# Autodesk Inventor assembly: Gantry
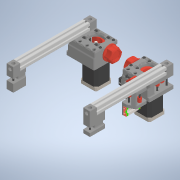
[picture p0: Inventor's stored thumbnail of the model, 180x180]
Saved by Autodesk Inventor 2022 (Build 260153000, 153)
## iProperties
Created: 2021-11-24
Part Number: Gantry
Document SubType Name: Assembly
Designer: yuto6
Author: yuto6
## Documents named in this file (7)
- C:\Users\yuto6\Documents\My3DPrinter\CAD\Asm\Gantry.iam
- C:\Users\yuto6\Documents\My3DPrinter\CAD\Parts\A_Idler (1).step.iam
- C:\Users\yuto6\Documents\My3DPrinter\CAD\Parts\B_Idler (1).step.iam
- C:\Users\yuto6\Documents\My3DPrinter\CAD\Parts\HFS3-1515-150.ipt
- C:\Users\yuto6\Documents\My3DPrinter\CAD\Parts\A_Drive.iam
- C:\Users\yuto6\Documents\My3DPrinter\CAD\Parts\B_Drive.iam
- C:\Users\yuto6\Documents\My3DPrinter\CAD\Parts\XY_Joint_Right.step.iam
## Components (7 placed, 6 different names)
1. B_Idler (1).step:1 [sub-assembly] — フラッシュ:1, フラッシュ:2, フラッシュ:3, メイト:1, メイト:2, メイト:5
2. A_Idler (1).step:1 [sub-assembly] — フラッシュ:1, フラッシュ:2, フラッシュ:4, メイト:3, メイト:4, メイト:5
3. HFS3-1515-150:1 — フラッシュ:3, メイト:1, メイト:2, メイト:8, メイト:9, フラッシュ:6
4. HFS3-1515-150:2 — フラッシュ:4, メイト:3, メイト:4, メイト:6, フラッシュ:5, メイト:7
5. A_Drive:1 [sub-assembly] — メイト:6, フラッシュ:5, メイト:7, フラッシュ:7, フラッシュ:8
6. B_Drive:1 [sub-assembly] — メイト:8, メイト:9, フラッシュ:6
7. XY_Joint_Right.step:1 [sub-assembly] — フラッシュ:7, フラッシュ:8
## Relationships (17: Mate 9, Flush 8)
- フラッシュ:1 [Flush]: B_Idler (1).step:1 ↔ A_Idler (1).step:1
- フラッシュ:2 [Flush]: B_Idler (1).step:1 ↔ A_Idler (1).step:1
- フラッシュ:3 [Flush]: B_Idler (1).step:1 ↔ HFS3-1515-150:1
- メイト:1 [Mate]: B_Idler (1).step:1 ↔ HFS3-1515-150:1
- メイト:2 [Mate]: B_Idler (1).step:1 ↔ HFS3-1515-150:1
- フラッシュ:4 [Flush]: A_Idler (1).step:1 ↔ HFS3-1515-150:2
- メイト:3 [Mate]: A_Idler (1).step:1 ↔ HFS3-1515-150:2
- メイト:4 [Mate]: A_Idler (1).step:1 ↔ HFS3-1515-150:2
- メイト:5 [Mate] (150 mm): B_Idler (1).step:1 ↔ A_Idler (1).step:1
- メイト:6 [Mate]: HFS3-1515-150:2 ↔ A_Drive:1
- フラッシュ:5 [Flush]: HFS3-1515-150:2 ↔ A_Drive:1
- メイト:7 [Mate]: HFS3-1515-150:2 ↔ A_Drive:1
- メイト:8 [Mate]: HFS3-1515-150:1 ↔ B_Drive:1
- メイト:9 [Mate]: HFS3-1515-150:1 ↔ B_Drive:1
- フラッシュ:6 [Flush]: HFS3-1515-150:1 ↔ B_Drive:1
- フラッシュ:7 [Flush] (1.2 mm): A_Drive:1 ↔ XY_Joint_Right.step:1
- フラッシュ:8 [Flush]: A_Drive:1 ↔ XY_Joint_Right.step:1
